# Autodesk Inventor assembly: assembly2
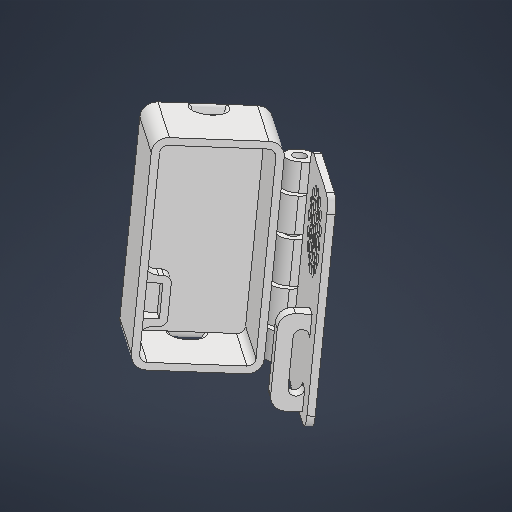
[picture p0: Inventor's stored thumbnail of the model, 512x512]
Saved by Autodesk Inventor 2026 (Build 300175050, 175E)
## iProperties
Created: 2025-05-28
Part Number: assembly2
Document SubType Name: Assembly
Designer: niall
Author: niall
## Documents named in this file (3)
- C:\Users\niall\My Files\UNI_UQ\2025_SEM_1\CSSE4011\Final Project\repo\wiki_assets\files\inventor\two\assembly2.iam
- C:\Users\niall\My Files\UNI_UQ\2025_SEM_1\CSSE4011\Final Project\repo\wiki_assets\files\inventor\two\box2.ipt
- C:\Users\niall\My Files\UNI_UQ\2025_SEM_1\CSSE4011\Final Project\repo\wiki_assets\files\inventor\two\lid2.ipt
## Components (2 placed, 2 different names)
1. box2:2 — Rotational:1
2. lid2:2 — Rotational:1
## Relationships (1: RevoluteJoint 1)
- Rotational:1 [RevoluteJoint] (22 mm): box2:2 ↔ lid2:2
